# Autodesk Inventor assembly: MG-Base Station PCB
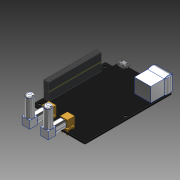
[picture p0: Inventor's stored thumbnail of the model, 180x180]
Saved by Autodesk Inventor 2019.4 (Build 234330000, 330)
## iProperties
Created: 2017-10-12
Part Number: MG-Base Station PCB
Document SubType Name: Assembly
Designer: ryll
Author: ryll
## Documents named in this file (7)
- D:\TIGERsGIT\Hardware\mechanik\2020\Inventor\Base Station\MG-Base Station PCB.iam
- D:\TIGERsGIT\Hardware\mechanik\2020\Inventor\Base Station\Base Station PCB.ipt
- D:\TIGERsGIT\Hardware\mechanik\2020\Inventor\Purchased Parts\Micro-USB.ipt
- D:\TIGERsGIT\Hardware\mechanik\2020\Inventor\Purchased Parts\RJ45 Socket.ipt
- D:\TIGERsGIT\Hardware\mechanik\2020\Inventor\Purchased Parts\Antenne-Klein.ipt
- D:\TIGERsGIT\Hardware\mechanik\2020\Inventor\Purchased Parts\SMA-F-RA.ipt
- D:\TIGERsGIT\Hardware\mechanik\2020\Inventor\Purchased Parts\ESQ-120-33-T-D\ESQ-120-33-T-D.iam
## Components (8 placed, 6 different names)
1. Base Station v3:1 — Passend:14, Passend:16, Fluchtend:4, Passend:17, Winkel:3, Passend:25, Passend:26, Passend:27, Passend:28, Passend:29, Passend:30, Fluchtend:7, Passend:31, Passend:32, Passend:33, Passend:34
2. Micro-USB 47346-0001:1 — Passend:14, Fluchtend:7, Passend:31
3. RJ45 Socket:1 — Passend:16, Fluchtend:4, Passend:17
4. Antenne-Klein:1 — Winkel:2, Einfügen:5
5. Antenne-Klein:2 — Winkel:2, Winkel:3, Einfügen:6
6. SMA-F-RA:1 — Passend:26, Passend:27, Passend:28, Einfügen:5
7. SMA-F-RA:2 — Passend:25, Passend:29, Passend:30, Einfügen:6
8. ESQ-120-33-T-D:1 [sub-assembly] — Passend:32, Passend:33, Passend:34
## Relationships (19: Mate 13, Flush 2, Angle 2, Insert 2)
- Passend:14 [Mate]: Base Station v3:1 ↔ Micro-USB 47346-0001:1
- Passend:16 [Mate]: Base Station v3:1 ↔ RJ45 Socket:1
- Fluchtend:4 [Flush] (-48.8 mm): Base Station v3:1 ↔ RJ45 Socket:1
- Passend:17 [Mate] (-75.9 mm): Base Station v3:1 ↔ RJ45 Socket:1
- Winkel:2 [Angle] (0 deg): Antenne-Klein:1 ↔ Antenne-Klein:2
- Winkel:3 [Angle] (0 deg): Base Station v3:1 ↔ Antenne-Klein:2
- Passend:25 [Mate]: Base Station v3:1 ↔ SMA-F-RA:2
- Passend:26 [Mate]: Base Station v3:1 ↔ SMA-F-RA:1
- Passend:27 [Mate] (-4 mm): Base Station v3:1 ↔ SMA-F-RA:1
- Passend:28 [Mate] (-19 mm): Base Station v3:1 ↔ SMA-F-RA:1
- Passend:29 [Mate] (-37 mm): Base Station v3:1 ↔ SMA-F-RA:2
- Passend:30 [Mate] (-4 mm): Base Station v3:1 ↔ SMA-F-RA:2
- Einfügen:5 [Insert] (3 mm): Antenne-Klein:1 ↔ SMA-F-RA:1
- Einfügen:6 [Insert] (3 mm): Antenne-Klein:2 ↔ SMA-F-RA:2
- Fluchtend:7 [Flush] (-12 mm): Base Station v3:1 ↔ Micro-USB 47346-0001:1
- Passend:31 [Mate] (-83.5 mm): Base Station v3:1 ↔ Micro-USB 47346-0001:1
- Passend:32 [Mate]: Base Station v3:1 ↔ ESQ-120-33-T-D:1
- Passend:33 [Mate] (-3.5 mm): Base Station v3:1 ↔ ESQ-120-33-T-D:1
- Passend:34 [Mate] (-42.5 mm): Base Station v3:1 ↔ ESQ-120-33-T-D:1
